# Autodesk Inventor assembly: UltibotsBed230x290
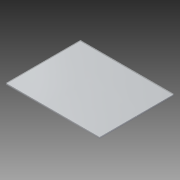
[picture p0: Inventor's stored thumbnail of the model, 180x180]
Saved by Autodesk Inventor 2015 SP1 (Build 190203100, 203)
## iProperties
Category: Misc
Created: 2014-12-22
Part Number: UltibotsBed230x290
Document SubType Name: Assembly
Designer: Jack
Mass: 752.15 g
Surface Area: 3728.19 cm^2
Volume: 334.095 cm^3
Density: 2.25131 g/cm^3
Vendor: Ultibots
Author: Jack
Title: Ultibots Bed 230x290
## Documents named in this file (4)
- C:\Users\Jack\ownCloud\Projects\CrossBot\InventorModel\HeatBed\Ultibots230x290\UltibotsBed230x290.iam
- C:\Users\Jack\ownCloud\Projects\CrossBot\InventorModel\HeatBed\Ultibots230x290\UltibotsGlass230x290.ipt
- C:\Users\Jack\ownCloud\Projects\CrossBot\InventorModel\HeatBed\Ultibots230x290\UltibotsKaptonHeater250x200.ipt
- C:\Users\Jack\ownCloud\Projects\CrossBot\InventorModel\HeatBed\Ultibots230x290\UltibotsHeatSpreader230x290.ipt
## Components (3 placed, 3 different names)
1. UltibotsGlass230x290:1 — Mate:1, Flush:1, Flush:2
2. UltibotsKaptonHeater250x200:1 — Mate:2, Flush:3, Flush:4
3. UltibotsHeatSpreader230x290:1 — Mate:1, Flush:1, Flush:2, Mate:2, Flush:3, Flush:4
## Relationships (6: Flush 4, Mate 2)
- Mate:1: UltibotsGlass230x290:1 ↔ UltibotsHeatSpreader230x290:1
- Flush:1 (0.5 mm): UltibotsGlass230x290:1 ↔ UltibotsHeatSpreader230x290:1
- Flush:2: UltibotsGlass230x290:1 ↔ UltibotsHeatSpreader230x290:1
- Mate:2: UltibotsKaptonHeater250x200:1 ↔ UltibotsHeatSpreader230x290:1
- Flush:3 (15 mm): UltibotsKaptonHeater250x200:1 ↔ UltibotsHeatSpreader230x290:1
- Flush:4 (20 mm): UltibotsKaptonHeater250x200:1 ↔ UltibotsHeatSpreader230x290:1
